# Autodesk Inventor assembly: modularRICH
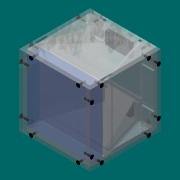
[picture p0: Inventor's stored thumbnail of the model, 180x180]
Saved by Autodesk Inventor 2016 (Build 200138000, 138)
## iProperties
Created: 2015-10-13
Part Number: modularRICH
Document SubType Name: Assembly
Designer: Sawaiz
Author: Sawaiz
## Documents named in this file (7)
- C:\Users\Sawaiz\OneDrive\projects\modularRICH\modularRICH.iam
- C:\Users\Sawaiz\OneDrive\projects\modularRICH\frame\frame.iam
- C:\Users\Sawaiz\OneDrive\projects\modularRICH\aerogelBlock.ipt
- C:\Users\Sawaiz\OneDrive\projects\modularRICH\fresnelLens.ipt
- C:\Users\Sawaiz\OneDrive\projects\modularRICH\mirror\mirrorSides.ipt
- C:\Users\Sawaiz\OneDrive\projects\modularRICH\mirror\topBottomMirror.iam
- C:\Users\Sawaiz\OneDrive\projects\modularRICH\modularRICH.xlsx
## Components (7 placed, 5 different names)
1. frame:1 [sub-assembly] — Mate:8, Mate:9, Mate:13, Mate:15, Mate:16, Mate:17, Flush:3, Flush:4, Flush:6, Mate:19, Mate:21, Mate:22, Flush:10, Flush:11
2. aerogelBlock:1 — Flush:8, Flush:9, Mate:23, Flush:10, Flush:11
3. fresnelLens:1 — Mate:19, Flush:8, Flush:9, Mate:23
4. mirrorSides:1 — Mate:8, Mate:9, Mate:21
5. mirrorSides:2 — Mate:13, Mate:15, Mate:22
6. topBottomMirror:1 [sub-assembly] — Mate:17, Flush:4, Flush:5, Flush:6
7. topBottomMirror:2 [sub-assembly] — Mate:16, Flush:3, Flush:5
## Relationships (18: Mate 10, Flush 8)
- Mate:8: frame:1 ↔ mirrorSides:1
- Mate:9: frame:1 ↔ mirrorSides:1
- Mate:13: frame:1 ↔ mirrorSides:2
- Mate:15: frame:1 ↔ mirrorSides:2
- Mate:16: frame:1 ↔ topBottomMirror:2
- Mate:17: frame:1 ↔ topBottomMirror:1
- Flush:3: frame:1 ↔ topBottomMirror:2
- Flush:4: frame:1 ↔ topBottomMirror:1
- Flush:5: topBottomMirror:1 ↔ topBottomMirror:2
- Flush:6 (30 mm): frame:1 ↔ topBottomMirror:1
- Mate:19: frame:1 ↔ fresnelLens:1
- Flush:8: aerogelBlock:1 ↔ fresnelLens:1
- Mate:21: frame:1 ↔ mirrorSides:1
- Mate:22: frame:1 ↔ mirrorSides:2
- Flush:9: aerogelBlock:1 ↔ fresnelLens:1
- Mate:23: aerogelBlock:1 ↔ fresnelLens:1
- Flush:10: frame:1 ↔ aerogelBlock:1
- Flush:11: frame:1 ↔ aerogelBlock:1
## Named parameters: acrylicThickness = 6.35 mm, aerogelThickness = 20 mm, height = 100 mm, width = 100 mm, depth = 100 mm, mirrorAngle = 17 deg, detectorWidth = 52 mm, detectorHeight = 52 mm, mirrorThickness = 3 mm, fresnelThickness = 0.1 mm, grooveDensity = 100, focalLength = 76.2 mm, ior = 1.49, centerThickness = 1.524 mm, fresnelAngle = 90 deg, fresnelEffectiveDiameter = 76.2 mm, mirrorSuppourtWidth = 40 mm
